# Autodesk Inventor assembly: Pickup 16
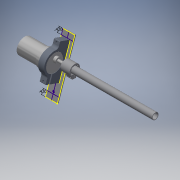
[picture p0: Inventor's stored thumbnail of the model, 180x180]
Saved by Autodesk Inventor 2017 (Build 210142000, 142)
## iProperties
Created: 2016-12-03
Part Number: Pickup 16
Document SubType Name: Assembly
Designer: Aditya
Author: Aditya
## Documents named in this file (7)
- C:\Users\Aditya\Documents\GitHub\RobotuxCAD\Team Robotux 15-16 Robot Cad Assets\Pickup 16.iam
- C:\Users\Aditya\Documents\GitHub\RobotuxCAD\Team Robotux 15-16 Robot Cad Assets\Tetrix Parts\tetrix_739089_2012.ipt
- C:\Users\Aditya\Documents\GitHub\RobotuxCAD\Team Robotux 15-16 Robot Cad Assets\pickup plate 1.ipt
- C:\Users\Aditya\Documents\GitHub\RobotuxCAD\Team Robotux 15-16 Robot Cad Assets\Part8.ipt
- C:\Users\Aditya\Documents\GitHub\RobotuxCAD\Team Robotux 15-16 Robot Cad Assets\tube_clamp_2012.ipt
- C:\Users\Aditya\Documents\GitHub\RobotuxCAD\Team Robotux 15-16 Robot Cad Assets\Tetrix Motor.ipt
- C:\Users\Aditya\Documents\GitHub\RobotuxCAD\Team Robotux 15-16 Robot Cad Assets\Tetrix Parts\tetrix_739079_collar_2012.ipt
## Components (6 placed, 6 different names)
1. tetrix_739089_2012:1 — Mate:11, Flush:2, Mate:12, Mate:13, Mate:14
2. Part8:1 — Mate:9, Mate:10
3. tube_clamp_2012:1 — Mate:6, Mate:7, Mate:8, Mate:9
4. Tetrix Motor:1 — Mate:5, Mate:6, Flush:1, Mate:10, Mate:11, Flush:2
5. tetrix_739079_collar_2012:1 — Mate:5, Mate:7, Mate:8, Flush:1
6. pickup plate 1:1 — Mate:12, Mate:13, Mate:14
## Relationships (12: Mate 10, Flush 2)
- Mate:5: Tetrix Motor:1 ↔ tetrix_739079_collar_2012:1
- Mate:6: tube_clamp_2012:1 ↔ Tetrix Motor:1
- Mate:7: tube_clamp_2012:1 ↔ tetrix_739079_collar_2012:1
- Mate:8: tube_clamp_2012:1 ↔ tetrix_739079_collar_2012:1
- Flush:1: Tetrix Motor:1 ↔ tetrix_739079_collar_2012:1
- Mate:9: Part8:1 ↔ tube_clamp_2012:1
- Mate:10: Part8:1 ↔ Tetrix Motor:1
- Mate:11: tetrix_739089_2012:1 ↔ Tetrix Motor:1
- Flush:2: tetrix_739089_2012:1 ↔ Tetrix Motor:1
- Mate:12: tetrix_739089_2012:1 ↔ pickup plate 1:1
- Mate:13: tetrix_739089_2012:1 ↔ pickup plate 1:1
- Mate:14: tetrix_739089_2012:1 ↔ pickup plate 1:1
